# Autodesk Inventor assembly: Сборка стрелялки
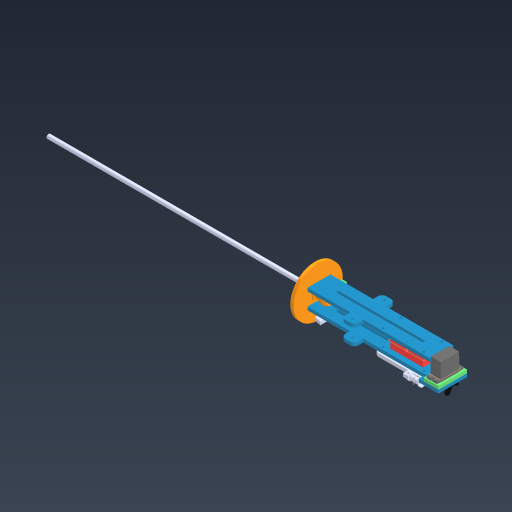
[picture p0: Inventor's stored thumbnail of the model, 512x512]
Saved by Autodesk Inventor 2023.2 (Build 272271030, 271C)
## iProperties
Created: 2023-12-17
Part Number: Сборка стрелялки
Document SubType Name: Assembly
Designer: I9232
Sending System: SolidWorks 2021
Last Author: liza
Last Saved: 2024-02-13
Author: I9232
## Documents named in this file (14)
- D:\!project\fox_n_crow_construction\crow\cheese_shooter\Сборка стрелялки\Сборка стрелялки.iam
- D:\!project\fox_n_crow_construction\crow\cheese_shooter\Сборка стрелялки\трубка.ipt
- D:\!project\fox_n_crow_construction\crow\cheese_shooter\Сборка стрелялки\крепежная деталь на трубку.ipt
- D:\!project\fox_n_crow_construction\crow\cheese_shooter\Сборка стрелялки\платформы держания.ipt
- D:\!project\fox_n_crow_construction\crow\cheese_shooter\Сборка стрелялки\платформы держания_2.ipt
- D:\!project\fox_n_crow_construction\crow\cheese_shooter\Сборка стрелялки\пружина.ipt
- D:\!project\fox_n_crow_construction\crow\cheese_shooter\Сборка стрелялки\боковая деталь.ipt
- D:\!project\fox_n_crow_construction\crow\cheese_shooter\Сборка стрелялки\боковая деталь_2.ipt
- D:\!project\fox_n_crow_construction\crow\cheese_shooter\Сборка стрелялки\MG90servo_assembly.iam
- D:\!project\fox_n_crow_construction\crow\cheese_shooter\Сборка стрелялки\направляющая.ipt
- D:\!project\fox_n_crow_construction\crow\cheese_shooter\Сборка стрелялки\вплавляющая втулка.ipt
- D:\!project\fox_n_crow_construction\crow\cheese_shooter\Сборка стрелялки\Деталь1^Сборка стрелялки.ipt
- D:\!project\fox_n_crow_construction\crow\cheese_shooter\Сборка стрелялки\M3x4.6x5.ipt
- D:\!project\fox_n_crow_construction\crow\cheese_shooter\Сборка стрелялки\Деталь9.ipt
## Components (13 placed, 11 different names)
1. трубка:1
2. крепежная деталь на трубку:1
3. платформы держания:1 — Симметрия:1
4. платформы держания:2 — Симметрия:1
5. пружина:1
6. боковая деталь:1
7. боковая деталь:3
8. MG90servo_assembly:1 [sub-assembly]
9. направляющая:1
10. вплавляющая втулка:4
11. Деталь1^Сборка стрелялки:1
12. M3x4.6x5:1
13. Деталь9:1
## Relationships (1: Symmetry 1)
- Симметрия:1 [Symmetry]: платформы держания:1 ↔ платформы держания:2
